# Autodesk Inventor assembly: femur +horn
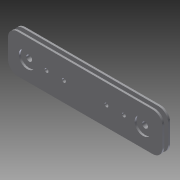
[picture p0: Inventor's stored thumbnail of the model, 180x180]
Saved by Autodesk Inventor 2012 (Build 160160000, 160)
## iProperties
Created: 2013-12-07
Part Number: femur +horn
Document SubType Name: Assembly
Designer: Irwan Haryanto
Author: Irwan Haryanto
## Documents named in this file (3)
- D:\Revenant\robot baru 2014\femur +horn.iam
- D:\Revenant\robot baru 2014\femur 6 cm.ipt
- D:\Revenant\robot baru 2014\Horn.ipt
## Components (4 placed, 2 different names)
1. femur 6 cm:1 — Insert:5, Insert:6, Insert:7, Insert:8
2. femur 6 cm:2 — Insert:1, Insert:2, Insert:3, Insert:4
3. Horn:1 — Insert:3, Insert:4, Insert:7, Insert:8
4. Horn:2 — Insert:1, Insert:2, Insert:5, Insert:6
## Relationships (8: Insert 8)
- Insert:1: femur 6 cm:2 ↔ Horn:2
- Insert:2: femur 6 cm:2 ↔ Horn:2
- Insert:3: femur 6 cm:2 ↔ Horn:1
- Insert:4: femur 6 cm:2 ↔ Horn:1
- Insert:5: femur 6 cm:1 ↔ Horn:2
- Insert:6: femur 6 cm:1 ↔ Horn:2
- Insert:7: femur 6 cm:1 ↔ Horn:1
- Insert:8: femur 6 cm:1 ↔ Horn:1
